# Autodesk Inventor assembly: dog_1
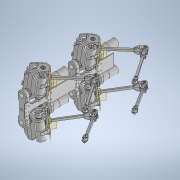
[picture p0: Inventor's stored thumbnail of the model, 180x180]
Saved by Autodesk Inventor 2020 (Build 240168000, 168)
## iProperties
Created: 2019-05-11
Part Number: dog_1
Document SubType Name: Assembly
Designer: psrob
Author: psrob
## Documents named in this file (7)
- E:\projects-2\project dog gen2\hardware\dog_1.iam
- E:\projects-2\project dog gen2\hardware\leg_ass_1.iam
- E:\projects-2\project dog gen2\hardware\leg_ass_1_MIR.iam
- E:\projects-2\project dog gen2\hardware\carbon_fiber_200.ipt
- E:\projects-2\project dog gen2\hardware\body_bone_1.ipt
- E:\projects-2\project dog gen2\hardware\body_bone_2.ipt
- E:\projects-2\project dog gen2\hardware\body_bone_3.ipt
## Components (9 placed, 6 different names)
1. leg_ass_1:1 [sub-assembly] — Flush:1, Mate:1, Flush:2, Flush:5, Flush:6, Flush:7, Flush:9, Flush:10, Insert:1, Angle:1, Insert:3, Tangent:4
2. leg_ass_1_MIR:1 [sub-assembly] — Flush:1, Mate:1, Flush:2, Flush:8, Mate:3, Insert:2, Mate:5, Tangent:3
3. leg_ass_1:2 [sub-assembly] — Flush:5, Flush:6, Flush:7, Mate:4, Tangent:1
4. leg_ass_1_MIR:2 [sub-assembly] — Tangent:2
5. carbon_fiber_200:1 — Flush:8, Flush:9, Mate:3
6. body_bone_1:1 — Flush:10, Insert:1, Angle:1
7. body_bone_2:1 — Insert:2, Insert:3
8. body_bone_3:1 — Mate:4, Tangent:1, Tangent:2
9. body_bone_1:2 — Mate:5, Tangent:3, Tangent:4
## Relationships (23: Flush 10, Mate 5, Tangent 4, Insert 3, Angle 1)
- Flush:1: leg_ass_1:1 ↔ leg_ass_1_MIR:1
- Mate:1: leg_ass_1:1 ↔ leg_ass_1_MIR:1
- Flush:2: leg_ass_1:1 ↔ leg_ass_1_MIR:1
- [Flush]: leg_ass_1:2 ↔ leg_ass_1_MIR:2
- [Mate]: leg_ass_1:2 ↔ leg_ass_1_MIR:2
- [Flush]: leg_ass_1:2 ↔ leg_ass_1_MIR:2
- Flush:5: leg_ass_1:1 ↔ leg_ass_1:2
- Flush:6: leg_ass_1:1 ↔ leg_ass_1:2
- Flush:7 (170 mm): leg_ass_1:1 ↔ leg_ass_1:2
- Flush:8 (5 mm): leg_ass_1_MIR:1 ↔ carbon_fiber_200:1
- Flush:9 (10 mm): leg_ass_1:1 ↔ carbon_fiber_200:1
- Mate:3 (-3 mm): leg_ass_1_MIR:1 ↔ carbon_fiber_200:1
- Flush:10: leg_ass_1:1 ↔ body_bone_1:1
- Insert:1: leg_ass_1:1 ↔ body_bone_1:1
- Angle:1 (0 deg): leg_ass_1:1 ↔ body_bone_1:1
- Insert:2: leg_ass_1_MIR:1 ↔ body_bone_2:1
- Insert:3: leg_ass_1:1 ↔ body_bone_2:1
- Mate:4: leg_ass_1:2 ↔ body_bone_3:1
- Tangent:1: leg_ass_1:2 ↔ body_bone_3:1
- Tangent:2: leg_ass_1_MIR:2 ↔ body_bone_3:1
- Mate:5: leg_ass_1_MIR:1 ↔ body_bone_1:2
- Tangent:3: leg_ass_1_MIR:1 ↔ body_bone_1:2
- Tangent:4: leg_ass_1:1 ↔ body_bone_1:2
## Named parameters: d10_d9 = 0 mm, d11_d7 = 0 mm, d12_d8 = 0 mm
